# Autodesk Inventor assembly: Lift.03.01.00.00
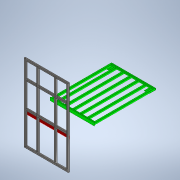
[picture p0: Inventor's stored thumbnail of the model, 180x180]
Saved by Autodesk Inventor 2021 (Build 250183000, 183)
## iProperties
_SolveAssemblyDoc: Frame Generator Solve Assembly
_Version: 25.0.0
Created: 2020-09-20
Part Number: Lift.03.01.00.00
Document SubType Name: Assembly
Designer: Kostya
Author: Kostya
## Documents named in this file (5)
- C:\Lift\Lift.03.01.00.00.iam
- C:\Lift\Lift.03.01.02.00.ipt
- C:\Lift\Lift.03.01.00.00\Frame\Frame 1600622124454.iam
- C:\Lift\Lift.03.01.01.00.iam
- C:\Lift\Lift.03.01.00.03.ipt
## Components (4 placed, 4 different names)
1. Lift.03.01.02.00:1
2. Frame 1600622124454:1 [sub-assembly] — Заподлицо:1, Совмещение:1, Заподлицо:3
3. Lift.03.01.01.00:1 [sub-assembly] — Заподлицо:1
4. Lift.03.01.00.03:1 — Совмещение:1, Заподлицо:3
## Relationships (3: Flush 2, Mate 1)
- Заподлицо:1 [Flush]: Frame 1600622124454:1 ↔ Lift.03.01.01.00:1
- Совмещение:1 [Mate]: Frame 1600622124454:1 ↔ Lift.03.01.00.03:1
- Заподлицо:3 [Flush]: Frame 1600622124454:1 ↔ Lift.03.01.00.03:1
